# Autodesk Inventor assembly: AR-100
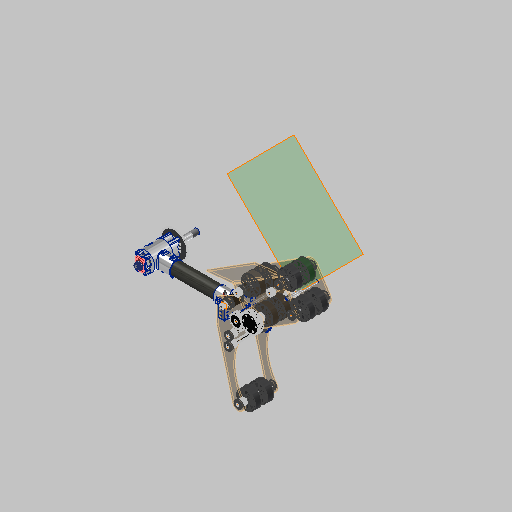
[picture p0: Inventor's stored thumbnail of the model, 512x512]
Saved by Autodesk Inventor 2023.5 (Build 275446000, 446)
## iProperties
Created: 2025-01-22
Part Number: AR-100
Document SubType Name: Assembly
Designer: slick
Mass: 2966.73 g
Surface Area: 9515.36 cm^2
Volume: 1838.81 cm^3
Author: slick
## Documents named in this file (15)
- C:\Users\slick\OneDrive\Desktop\2025-ReefScape---CAD\Arm\AR-100.iam
- C:\Users\slick\OneDrive\Desktop\2025-ReefScape---CAD\Arm\AR-001.ipt
- C:\Users\slick\OneDrive\Desktop\2025-ReefScape---CAD\COMMON PARTS\BEARINGS\0_875_ID_x_1_875_OD_X_0_500_Radial_Bearing_EE11S-2RS.ipt
- C:\Users\slick\OneDrive\Desktop\2025-ReefScape---CAD\Arm\AR-005.ipt
- C:\Users\slick\OneDrive\Desktop\2025-ReefScape---CAD\Arm\AR-006.ipt
- C:\Users\slick\OneDrive\Desktop\2025-ReefScape---CAD\COMMON PARTS\SPROCKETS\35\WCP-0983\WCP-0983.ipt
- C:\Users\slick\OneDrive\Desktop\2025-ReefScape---CAD\Arm\AR-009.ipt
- C:\Users\slick\OneDrive\Desktop\2025-ReefScape---CAD\Arm\AR-010.ipt
- C:\Users\slick\OneDrive\Desktop\2025-ReefScape---CAD\Gripper\GP3\GP3-100.iam
- C:\Users\slick\OneDrive\Desktop\2025-ReefScape---CAD\Gripper\GP4\GP4-100.iam
- C:\Users\slick\OneDrive\Desktop\2025-ReefScape---CAD\Arm\AR-013.ipt
- C:\Users\slick\OneDrive\Desktop\2025-ReefScape---CAD\Arm\AR-014.ipt
- C:\Users\slick\OneDrive\Desktop\2025-ReefScape---CAD\Elevator\EL2\EL2-A-012.ipt
- C:\Users\slick\OneDrive\Desktop\2025-ReefScape---CAD\Arm\AR-015.ipt
- C:\Users\slick\OneDrive\Desktop\2025-ReefScape---CAD\COMMON PARTS\SDS MK4i Swerve Module, 10-32, Falcons\CANcoder Assembly.iam
## Components (15 placed, 14 different names)
1. AR-001:1 — Mate:1, Mate:2, Mate:3, Mate:4, Mate:13, Mate:14, Insert:37, Insert:38, Insert:39, Insert:40
2. 0_875_ID_x_1_875_OD_X_0_500_Radial_Bearing_EE11S-2RS:1 — Mate:1, Mate:3, Mate:15, Flush:2, Mate:20
3. 0_875_ID_x_1_875_OD_X_0_500_Radial_Bearing_EE11S-2RS:2 — Mate:2, Mate:4
4. AR-005:1 — Mate:13, Mate:14, Mate:17, Mate:18
5. AR-006:1 — Mate:15, Flush:2, Insert:36, Mate:19, Angle:1
6. WCP-0983:1 — Insert:21, Insert:22, Insert:23, Insert:24
7. AR-009:1 — Insert:21, Insert:22, Insert:23, Insert:24, Insert:39, Insert:40
8. AR-010:1 — Mate:17, Mate:18, Insert:25, Insert:26, Insert:34, Insert:35
9. GP3-100:1 [sub-assembly] — Insert:25, Insert:26
10. GP4-100:1 [sub-assembly] — Insert:34, Insert:35, Angle:1
11. AR-013:1 — Insert:36
12. AR-014:1 — Insert:37, Insert:38, Insert:41, Insert:42
13. EL2-A-012:1 — Mate:19, Mate:20
14. AR-015:1 — Insert:41, Insert:42, Insert:43, Insert:44
15. CANcoder Assembly:1 [sub-assembly] — Insert:43, Insert:44
## Relationships (30: Insert 17, Mate 11, Flush 1, Angle 1)
- Mate:1: AR-001:1 ↔ 0_875_ID_x_1_875_OD_X_0_500_Radial_Bearing_EE11S-2RS:1
- Mate:2: AR-001:1 ↔ 0_875_ID_x_1_875_OD_X_0_500_Radial_Bearing_EE11S-2RS:2
- Mate:3: AR-001:1 ↔ 0_875_ID_x_1_875_OD_X_0_500_Radial_Bearing_EE11S-2RS:1
- Mate:4: AR-001:1 ↔ 0_875_ID_x_1_875_OD_X_0_500_Radial_Bearing_EE11S-2RS:2
- Mate:13: AR-001:1 ↔ AR-005:1
- Mate:14 (-50.8 mm): AR-001:1 ↔ AR-005:1
- Mate:15: 0_875_ID_x_1_875_OD_X_0_500_Radial_Bearing_EE11S-2RS:1 ↔ AR-006:1
- Flush:2 (-12.7 mm): 0_875_ID_x_1_875_OD_X_0_500_Radial_Bearing_EE11S-2RS:1 ↔ AR-006:1
- Insert:21: WCP-0983:1 ↔ AR-009:1
- Insert:22: WCP-0983:1 ↔ AR-009:1
- Insert:23: WCP-0983:1 ↔ AR-009:1
- Insert:24: WCP-0983:1 ↔ AR-009:1
- Mate:17: AR-005:1 ↔ AR-010:1
- Mate:18: AR-005:1 ↔ AR-010:1
- Insert:25: AR-010:1 ↔ GP3-100:1
- Insert:26: AR-010:1 ↔ GP3-100:1
- Insert:34: AR-010:1 ↔ GP4-100:1
- Insert:35: AR-010:1 ↔ GP4-100:1
- Insert:36: AR-006:1 ↔ AR-013:1
- Insert:37: AR-001:1 ↔ AR-014:1
- Insert:38: AR-001:1 ↔ AR-014:1
- Insert:39: AR-001:1 ↔ AR-009:1
- Insert:40: AR-001:1 ↔ AR-009:1
- Mate:19: AR-006:1 ↔ EL2-A-012:1
- Mate:20: 0_875_ID_x_1_875_OD_X_0_500_Radial_Bearing_EE11S-2RS:1 ↔ EL2-A-012:1
- Insert:41: AR-014:1 ↔ AR-015:1
- Insert:42: AR-014:1 ↔ AR-015:1
- Insert:43: AR-015:1 ↔ CANcoder Assembly:1
- Insert:44: AR-015:1 ↔ CANcoder Assembly:1
- Angle:1 (0 deg): AR-006:1 ↔ GP4-100:1
